# Autodesk Inventor assembly: Back_Pane_Basel_Assembly
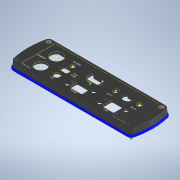
[picture p0: Inventor's stored thumbnail of the model, 180x180]
Saved by Autodesk Inventor 2022 (Build 260153000, 153)
## iProperties
Created: 2020-07-14
Part Number: Back_Pane_Basel_Assembly
Document SubType Name: Assembly
Designer: CASE-SMALL2
Author: CASE-SMALL2
## Documents named in this file (5)
- D:\Drive\Chalmers\Fortsatt arbete WR\Design files\GPS Base Station\Back_Panel\Panel\Back_Panel_Base_Assembly.iam
- D:\Drive\Chalmers\Fortsatt arbete WR\Design files\GPS Base Station\Back_Panel\Panel\1009799_3D_Back.ipt
- D:\Drive\Chalmers\Fortsatt arbete WR\Design files\GPS Base Station\Back_Panel\Panel\DI 1600.ipt
- D:\Drive\Chalmers\Fortsatt arbete WR\Design files\GPS Base Station\Back_Panel\Panel\SHR Z KT30X10 WN 1452 OG_3DSYM.ipt
- D:\Drive\Chalmers\Fortsatt arbete WR\Design files\GPS Base Station\Back_Panel\Panel\1009410_3D.ipt
## Components (8 placed, 4 different names)
1. 1009799_3D_Back:1 — Rigid:1, Rigid:2, Rigid:3, Rigid:4, Rigid:6, Rigid:9, Rigid:10
2. DI 1600:1 — Rigid:10
3. SHR Z KT30X10 WN 1452 OG_3DSYM:1 — Rigid:1
4. SHR Z KT30X10 WN 1452 OG_3DSYM:2 — Rigid:3
5. SHR Z KT30X10 WN 1452 OG_3DSYM:3 — Rigid:4
6. SHR Z KT30X10 WN 1452 OG_3DSYM:4 — Rigid:2
7. 1009410_3D:1 — Rigid:6
8. 1009410_3D:2 — Rigid:9
## Relationships (7: WeldJoint 7)
- Rigid:1 [WeldJoint]: 1009799_3D_Back:1 ↔ SHR Z KT30X10 WN 1452 OG_3DSYM:1
- Rigid:2 [WeldJoint]: 1009799_3D_Back:1 ↔ SHR Z KT30X10 WN 1452 OG_3DSYM:4
- Rigid:3 [WeldJoint]: 1009799_3D_Back:1 ↔ SHR Z KT30X10 WN 1452 OG_3DSYM:2
- Rigid:4 [WeldJoint]: 1009799_3D_Back:1 ↔ SHR Z KT30X10 WN 1452 OG_3DSYM:3
- Rigid:6 [WeldJoint]: 1009799_3D_Back:1 ↔ 1009410_3D:1
- Rigid:9 [WeldJoint]: 1009799_3D_Back:1 ↔ 1009410_3D:2
- Rigid:10 [WeldJoint]: 1009799_3D_Back:1 ↔ DI 1600:1
